# Autodesk Inventor assembly: Track Frame Assembly
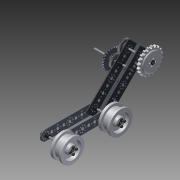
[picture p0: Inventor's stored thumbnail of the model, 180x180]
Saved by Autodesk Inventor 2015 (Build 190159000, 159)
## iProperties
Created: 2015-09-27
Part Number: Track Frame Assembly
Document SubType Name: Assembly
Designer: Jing-Chen
Author: Jing-Chen
## Documents named in this file (15)
- C:\Users\Jing-Chen\Desktop\Bionic Hybrids 2016\Bionic-Hybrids\CAD\Drivetrain\Sub-Assemblies\Track Frame Assembly.iam
- C:\Users\Jing-Chen\Desktop\Bionic Hybrids 2016\Bionic-Hybrids\Stock\Bracket-U9 - 739067.ipt
- C:\Users\Jing-Chen\Desktop\Bionic Hybrids 2016\Bionic-Hybrids\CAD\Drivetrain\Sub-Assemblies\Track Idler Assembly.iam
- C:\Users\Jing-Chen\Desktop\Bionic Hybrids 2016\Bionic-Hybrids\Stock\Bearing-Thrust - 739091.ipt
- C:\Users\Jing-Chen\Desktop\Bionic Hybrids 2016\Bionic-Hybrids\Stock\Shaft Collar-Setscrew, Axle - 739092.iam
- C:\Users\Jing-Chen\Desktop\Bionic Hybrids 2016\Bionic-Hybrids\Stock\Track Sprocket - 736468.ipt
- C:\Users\Jing-Chen\Desktop\Bionic Hybrids 2016\Bionic-Hybrids\Stock\Shaft Collar-Setscrew, Axle, Mountable - 739172.iam
- C:\Users\Jing-Chen\Desktop\Bionic Hybrids 2016\Bionic-Hybrids\Stock\Plate-9x1 - 739272.ipt
- C:\Users\Jing-Chen\Desktop\Bionic Hybrids 2016\Bionic-Hybrids\Stock\Spacer 3.125mm- 739100.ipt
- C:\Users\Jing-Chen\Desktop\Bionic Hybrids 2016\Bionic-Hybrids\Stock\Gear-40 tooth - 731901.ipt
- C:\Users\Jing-Chen\Desktop\Bionic Hybrids 2016\Bionic-Hybrids\Stock\Plate-1x1 - 739387.ipt
- C:\Users\Jing-Chen\Desktop\Bionic Hybrids 2016\Bionic-Hybrids\Stock\Screw 0.5in - 739097.ipt
- C:\Users\Jing-Chen\Desktop\Bionic Hybrids 2016\Bionic-Hybrids\CAD\Drivetrain\Modified Parts\Cut 100mm axle.ipt
- C:\Users\Jing-Chen\Desktop\Bionic Hybrids 2016\Bionic-Hybrids\CAD\Drivetrain\Sub-Assemblies\Tread Sprocket Assembly.iam
- C:\Users\Jing-Chen\Desktop\Bionic Hybrids 2016\Bionic-Hybrids\Stock\Axle-100mm - 739088.ipt
## Components (33 placed, 14 different names)
1. Bracket-U9 - 739067:1 — Mate:16, Mate:17, Mate:18, Mate:19, Mate:20, Mate:21, Mate:44, Mate:46, Mate:60, Mate:61, Mate:63, Mate:66, Mate:67, Mate:88, Mate:89, Mate:90, Mate:91, Mate:108, Mate:122
2. Track Idler Assembly:1 [sub-assembly] — Mate:43, Flush:9, Mate:134
3. Shaft Collar-Setscrew, Axle - 739092:1 [sub-assembly] — Mate:42, Mate:133
4. Track Sprocket - 736468:1 — Mate:13, Mate:15, Mate:105, Mate:126
5. Shaft Collar-Setscrew, Axle, Mountable - 739172:1 [sub-assembly] — Mate:13, Mate:15, Mate:105, Mate:106, Mate:109, Angle:5
6. Plate-9x1 - 739272:1 — Mate:16, Mate:19, Mate:21, Mate:37, Mate:38, Mate:45, Flush:4, Flush:5, Mate:53
7. Plate-9x1 - 739272:2 — Mate:17, Mate:18, Mate:20, Mate:39, Mate:40, Mate:47
8. Cut 100mm axle:1 — Mate:107, Angle:4, Mate:109, Angle:5, Mate:121, Mate:124, Mate:125, Flush:7
9. Bearing-Thrust - 739091:5 — Mate:44, Mate:45, Mate:50, Mate:129
10. Bearing-Thrust - 739091:6 — Mate:39, Mate:40, Mate:42, Mate:132
11. Bearing-Thrust - 739091:10 — Mate:46, Mate:47, Mate:52
12. Bearing-Thrust - 739091:11 — Mate:37, Mate:38, Mate:43
13. Cut 100mm axle:2 — Mate:129, Flush:8, Mate:130, Mate:131
14. Track Idler Assembly:2 [sub-assembly] — Mate:50, Flush:8, Mate:130
15. Shaft Collar-Setscrew, Axle - 739092:2 [sub-assembly] — Mate:52, Mate:131
16. Gear-40 tooth - 731901:1 — Mate:55, Mate:57, Mate:64, Mate:84, Mate:85, Mate:86, Mate:87, Rotation:1
17. Shaft Collar-Setscrew, Axle, Mountable - 739172:2 [sub-assembly] — Mate:55, Mate:57, Mate:63, Mate:64, Mate:107, Mate:108, Angle:4
18. Shaft Collar-Setscrew, Axle, Mountable - 739172:4 [sub-assembly] — Mate:60, Mate:61, Mate:66, Angle:1
19. Axle-100mm - 739088:1 — Angle:1
20. Plate-1x1 - 739387:1 — Mate:67, Mate:70
21. Bearing-Thrust - 739091:12 — Mate:70, Mate:72
22. Spacer 3.125mm- 739100:3 — Mate:72, Mate:128
23. Screw 0.5in - 739097:1 — Mate:84, Mate:86
24. Screw 0.5in - 739097:2 — Mate:85, Mate:87
25. Screw 0.5in - 739097:3 — Mate:88, Mate:90
26. Screw 0.5in - 739097:4 — Mate:89, Mate:91
27. Spacer 3.125mm- 739100:5 — Mate:102, Mate:123, Mate:124
28. Spacer 3.125mm- 739100:6 — Mate:102, Mate:103
29. Spacer 3.125mm- 739100:7 — Mate:103, Mate:106
30. Bearing-Thrust - 739091:13 — Mate:121, Mate:122, Mate:123
31. Bearing-Thrust - 739091:14 — Mate:125, Mate:126, Flush:7
32. Tread Sprocket Assembly:1 [sub-assembly] — Mate:128, Rotation:1
33. Cut 100mm axle:3 — Flush:9, Mate:132, Mate:133, Mate:134
## Relationships (85: Mate 72, Flush 7, Angle 5, RelateRotation 1)
- Mate:13: Track Sprocket - 736468:1 ↔ Shaft Collar-Setscrew, Axle, Mountable - 739172:1
- Mate:15: Track Sprocket - 736468:1 ↔ Shaft Collar-Setscrew, Axle, Mountable - 739172:1
- Mate:16: Bracket-U9 - 739067:1 ↔ Plate-9x1 - 739272:1
- Mate:17: Bracket-U9 - 739067:1 ↔ Plate-9x1 - 739272:2
- Mate:18: Bracket-U9 - 739067:1 ↔ Plate-9x1 - 739272:2
- Mate:19: Bracket-U9 - 739067:1 ↔ Plate-9x1 - 739272:1
- Mate:20: Bracket-U9 - 739067:1 ↔ Plate-9x1 - 739272:2
- Mate:21: Bracket-U9 - 739067:1 ↔ Plate-9x1 - 739272:1
- [Mate]: Shaft Collar-Setscrew, Axle, Mountable - 739172:1 ↔ Cut 100mm axle:1
- Mate:37: Plate-9x1 - 739272:1 ↔ Bearing-Thrust - 739091:11
- Mate:38: Plate-9x1 - 739272:1 ↔ Bearing-Thrust - 739091:11
- Mate:39: Plate-9x1 - 739272:2 ↔ Bearing-Thrust - 739091:6
- Mate:40: Plate-9x1 - 739272:2 ↔ Bearing-Thrust - 739091:6
- Mate:42: Shaft Collar-Setscrew, Axle - 739092:1 ↔ Bearing-Thrust - 739091:6
- Mate:43: Track Idler Assembly:1 ↔ Bearing-Thrust - 739091:11
- Mate:44: Bracket-U9 - 739067:1 ↔ Bearing-Thrust - 739091:5
- Mate:45: Plate-9x1 - 739272:1 ↔ Bearing-Thrust - 739091:5
- Mate:46: Bracket-U9 - 739067:1 ↔ Bearing-Thrust - 739091:10
- Mate:47: Plate-9x1 - 739272:2 ↔ Bearing-Thrust - 739091:10
- [Mate]: Bearing-Thrust - 739091:5 ↔ Cut 100mm axle:2
- [Mate]: Cut 100mm axle:2 ↔ Track Idler Assembly:2
- Mate:50: Bearing-Thrust - 739091:5 ↔ Track Idler Assembly:2
- [Flush]: Cut 100mm axle:2 ↔ Track Idler Assembly:2
- [Mate]: Cut 100mm axle:2 ↔ Shaft Collar-Setscrew, Axle - 739092:2
- Mate:52: Bearing-Thrust - 739091:10 ↔ Shaft Collar-Setscrew, Axle - 739092:2
- Flush:4: Plate-9x1 - 739272:1
- Flush:5: Plate-9x1 - 739272:1
- Mate:53: Plate-9x1 - 739272:1
- Mate:55: Gear-40 tooth - 731901:1 ↔ Shaft Collar-Setscrew, Axle, Mountable - 739172:2
- Mate:57: Gear-40 tooth - 731901:1 ↔ Shaft Collar-Setscrew, Axle, Mountable - 739172:2
- [Mate]: Cut 100mm axle:1 ↔ Shaft Collar-Setscrew, Axle, Mountable - 739172:2
- Mate:60: Bracket-U9 - 739067:1 ↔ Shaft Collar-Setscrew, Axle, Mountable - 739172:4
- Mate:61: Bracket-U9 - 739067:1 ↔ Shaft Collar-Setscrew, Axle, Mountable - 739172:4
- Mate:63: Bracket-U9 - 739067:1 ↔ Shaft Collar-Setscrew, Axle, Mountable - 739172:2
- Mate:64: Gear-40 tooth - 731901:1 ↔ Shaft Collar-Setscrew, Axle, Mountable - 739172:2
- [Mate]: Shaft Collar-Setscrew, Axle, Mountable - 739172:4 ↔ Axle-100mm - 739088:1
- [Flush]: Shaft Collar-Setscrew, Axle, Mountable - 739172:4 ↔ Axle-100mm - 739088:1
- Mate:66: Bracket-U9 - 739067:1 ↔ Shaft Collar-Setscrew, Axle, Mountable - 739172:4
- Mate:67: Bracket-U9 - 739067:1 ↔ Plate-1x1 - 739387:1
- [Mate]: Axle-100mm - 739088:1 ↔ Plate-1x1 - 739387:1
- [Mate]: Axle-100mm - 739088:1 ↔ Bearing-Thrust - 739091:12
- Mate:70: Plate-1x1 - 739387:1 ↔ Bearing-Thrust - 739091:12
- [Mate]: Axle-100mm - 739088:1 ↔ Spacer 3.125mm- 739100:3
- Mate:72: Bearing-Thrust - 739091:12 ↔ Spacer 3.125mm- 739100:3
- Angle:1 (180 deg): Shaft Collar-Setscrew, Axle, Mountable - 739172:4 ↔ Axle-100mm - 739088:1
- Mate:84: Gear-40 tooth - 731901:1 ↔ Screw 0.5in - 739097:1
- Mate:85: Gear-40 tooth - 731901:1 ↔ Screw 0.5in - 739097:2
- Mate:86: Gear-40 tooth - 731901:1 ↔ Screw 0.5in - 739097:1
- Mate:87: Gear-40 tooth - 731901:1 ↔ Screw 0.5in - 739097:2
- Mate:88: Bracket-U9 - 739067:1 ↔ Screw 0.5in - 739097:3
- Mate:89: Bracket-U9 - 739067:1 ↔ Screw 0.5in - 739097:4
- Mate:90: Bracket-U9 - 739067:1 ↔ Screw 0.5in - 739097:3
- Mate:91: Bracket-U9 - 739067:1 ↔ Screw 0.5in - 739097:4
- [Mate]: Cut 100mm axle:1 ↔ Spacer 3.125mm- 739100:7
- [Mate]: Cut 100mm axle:1 ↔ Spacer 3.125mm- 739100:6
- [Mate]: Cut 100mm axle:1 ↔ Spacer 3.125mm- 739100:5
- Mate:102: Spacer 3.125mm- 739100:5 ↔ Spacer 3.125mm- 739100:6
- Mate:103: Spacer 3.125mm- 739100:6 ↔ Spacer 3.125mm- 739100:7
- Mate:105: Track Sprocket - 736468:1 ↔ Shaft Collar-Setscrew, Axle, Mountable - 739172:1
- Mate:106: Shaft Collar-Setscrew, Axle, Mountable - 739172:1 ↔ Spacer 3.125mm- 739100:7
- [Angle] (180 deg): Cut 100mm axle:1 ↔ Shaft Collar-Setscrew, Axle, Mountable - 739172:2
- [Angle] (180 deg): Shaft Collar-Setscrew, Axle, Mountable - 739172:1 ↔ Cut 100mm axle:1
- Mate:107: Cut 100mm axle:1 ↔ Shaft Collar-Setscrew, Axle, Mountable - 739172:2
- Mate:108: Bracket-U9 - 739067:1 ↔ Shaft Collar-Setscrew, Axle, Mountable - 739172:2
- Angle:4 (180 deg): Cut 100mm axle:1 ↔ Shaft Collar-Setscrew, Axle, Mountable - 739172:2
- Mate:109: Shaft Collar-Setscrew, Axle, Mountable - 739172:1 ↔ Cut 100mm axle:1
- Angle:5 (180 deg): Shaft Collar-Setscrew, Axle, Mountable - 739172:1 ↔ Cut 100mm axle:1
- Mate:121: Cut 100mm axle:1 ↔ Bearing-Thrust - 739091:13
- Mate:122: Bracket-U9 - 739067:1 ↔ Bearing-Thrust - 739091:13
- Mate:123: Spacer 3.125mm- 739100:5 ↔ Bearing-Thrust - 739091:13
- Mate:124: Cut 100mm axle:1 ↔ Spacer 3.125mm- 739100:5
- Mate:125: Cut 100mm axle:1 ↔ Bearing-Thrust - 739091:14
- Mate:126: Track Sprocket - 736468:1 ↔ Bearing-Thrust - 739091:14
- Flush:7: Cut 100mm axle:1 ↔ Bearing-Thrust - 739091:14
- [Mate]: Axle-100mm - 739088:1 ↔ Tread Sprocket Assembly:1
- Mate:128: Spacer 3.125mm- 739100:3 ↔ Tread Sprocket Assembly:1
- Rotation:1 [RelateRotation] (1 ul): Gear-40 tooth - 731901:1 ↔ Tread Sprocket Assembly:1
- Mate:129: Bearing-Thrust - 739091:5 ↔ Cut 100mm axle:2
- Flush:8: Cut 100mm axle:2 ↔ Track Idler Assembly:2
- Mate:130: Cut 100mm axle:2 ↔ Track Idler Assembly:2
- Mate:131: Cut 100mm axle:2 ↔ Shaft Collar-Setscrew, Axle - 739092:2
- Flush:9: Track Idler Assembly:1 ↔ Cut 100mm axle:3
- Mate:132: Bearing-Thrust - 739091:6 ↔ Cut 100mm axle:3
- Mate:133: Shaft Collar-Setscrew, Axle - 739092:1 ↔ Cut 100mm axle:3
- Mate:134: Track Idler Assembly:1 ↔ Cut 100mm axle:3
